# Autodesk Inventor assembly: GPS-Compass_assembly
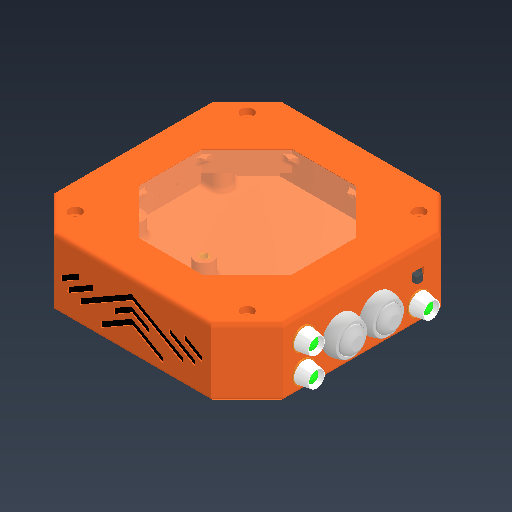
[picture p0: Inventor's stored thumbnail of the model, 512x512]
Saved by Autodesk Inventor 2026.2 (Build 302298000, 298)
## iProperties
Created: 2025-11-19
Part Number: GPS-Compass_assembly
Document SubType Name: Assembly
Designer: MenMe
Author: MenMe
## Documents named in this file (15)
- C:\Users\MenMe\Documents\GitHub\GPS-Compass\_mechanical\GPS-Compass_assembly\GPS-Compass_assembly.iam
- C:\Users\MenMe\Documents\GitHub\GPS-Compass\_mechanical\GPS-Compass_assembly\GPS-Compass_box.ipt
- C:\Users\MenMe\Documents\GitHub\GPS-Compass\_mechanical\GPS-Compass_assembly\GPS-Compass_top.ipt
- C:\Users\MenMe\Documents\GitHub\GPS-Compass\_mechanical\GPS-Compass_assembly\GPS-Compass_plexi.ipt
- C:\Users\MenMe\Documents\GitHub\GPS-Compass\_mechanical\GPS-Compass_assembly\parts\DODGE INSERT M3X4(D5-Dill4.8)\DODGE INSERT M3X4(D5-Dill4.8)\DODGE INSERT M3X4(D5-Dill4.8).ipt
- C:\Users\MenMe\Documents\GitHub\GPS-Compass\_mechanical\GPS-Compass_assembly\parts\ic184-thread\ic184-thread\ic184-thread.ipt
- C:\Users\MenMe\Documents\GitHub\GPS-Compass\_mechanical\GPS-Compass_assembly\parts\Copper Shell LED Indicator Light KL0624\Copper Shell LED Indicator Light KL0624\Copper Shell LED Indicator Light KL0624.ipt
- C:\Users\MenMe\Documents\GitHub\GPS-Compass\_mechanical\GPS-Compass_assembly\parts\EG1201\EG1201\EG1201.ipt
- C:\Users\MenMe\Documents\GitHub\GPS-Compass\_mechanical\GPS-Compass_assembly\parts\antena\antena\antena.ipt
- C:\Users\MenMe\Documents\GitHub\GPS-Compass\_mechanical\PCB_3D_models\GPS-Compass\GPS-Compass\GPS-Compass.ipt
- C:\Users\MenMe\Documents\GitHub\GPS-Compass\_mechanical\PCB_3D_models\GPS-Compass_UI\GPS-Compass_UI\GPS-Compass_UI.ipt
- C:\Users\MenMe\Documents\GitHub\GPS-Compass\_mechanical\PCB_3D_models\GPS-Compass_GNSS\GPS-Compass_GNSS\GPS-Compass_GNSS.ipt
- C:\Users\MenMe\Documents\GitHub\GPS-Compass\_mechanical\PCB_3D_models\GPS-Compass_Arrow\GPS-Compass_Arrow\GPS-Compass_Arrow.ipt
- C:\Users\MenMe\Documents\Inventor\Content Center Files\R2026\en-US\ISO 4762(2)\ISO 4762 - M3 x 12ISO.ipt
- C:\Users\MenMe\Documents\Inventor\Content Center Files\R2026\en-US\ISO 4762(2)\ISO 4762 - M3 x 6ISO.ipt
## Components (36 placed, 14 different names)
1. GPS-Compass_box:1 — Insert:7, Insert:8, Insert:9, Mate:11, Insert:10, Insert:12, Insert:15, Insert:21, Flush:5, Flush:6, Flush:7, Insert:48, Insert:49, Insert:50, Mate:28, Mate:30, Mate:32, Insert:64, Insert:65, Mate:33, Mate:34, Insert:66, Insert:67
2. GPS-Compass_top:1 — Mate:8, Flush:5, Flush:6, Flush:7, Mate:17, Insert:51, Insert:52, Insert:53, Insert:54, Insert:55, Insert:56, Mate:28, Mate:29
3. GPS-Compass_plexi:1 — Mate:8, Mate:17, Mate:29
4. GPS-Compass:1 — Flush:8, Flush:9, Mate:26, Flush:10, Flush:11, Mate:27, Insert:49, Insert:50, Insert:57, Insert:58, Insert:60, Insert:62, Insert:63
5. GPS-Compass_UI:1 — Flush:8, Flush:9, Mate:26
6. GPS-Compass_GNSS:1 — Flush:10, Flush:11, Mate:27, Insert:59, Insert:61
7. GPS-Compass_Arrow:1 — Insert:51, Insert:52
8. Copper Shell LED Indicator Light KL0624:1 — Insert:48
9. EG1201:1 — Mate:30, Mate:32
10. antena:1 — Mate:33, Mate:34
11. ic184-thread:4 — Insert:64
12. ic184-thread:5 — Insert:65
13. Copper Shell LED Indicator Light KL0624:2 — Insert:67
14. Copper Shell LED Indicator Light KL0624:3 — Insert:66
15. ISO 4762 M3 x 12:1 — Insert:53
16. ISO 4762 M3 x 12:2 — Insert:54
17. ISO 4762 M3 x 12:4 — Insert:55
18. ISO 4762 M3 x 12:5 — Insert:56
19. ISO 4762 M3 x 6:1 — Insert:57
20. ISO 4762 M3 x 6:2 — Insert:58
21. ISO 4762 M3 x 6:3 — Insert:59
22. ISO 4762 M3 x 6:4 — Insert:61
23. ISO 4762 M3 x 6:5 — Insert:62
24. ISO 4762 M3 x 6:7 — Insert:63
25. ISO 4762 M3 x 6:8 — Insert:60
26. DODGE INSERT M3X4(D5-Dill4.8):3 — Insert:7
27. DODGE INSERT M3X4(D5-Dill4.8):4 — Insert:8
28. DODGE INSERT M3X4(D5-Dill4.8):5 — Insert:9
29. DODGE INSERT M3X4(D5-Dill4.8):6 — Mate:11
30. DODGE INSERT M3X4(D5-Dill4.8):7 — Insert:10
31. DODGE INSERT M3X4(D5-Dill4.8):9 — Insert:12
32. DODGE INSERT M3X4(D5-Dill4.8):12 — Insert:15
33. DODGE INSERT M3X4(D5-Dill4.8):13
34. DODGE INSERT M3X4(D5-Dill4.8):14
35. DODGE INSERT M3X4(D5-Dill4.8):15
36. DODGE INSERT M3X4(D5-Dill4.8):16 — Insert:21
## Relationships (45: Insert 27, Mate 11, Flush 7)
- Mate:8: GPS-Compass_top:1 ↔ GPS-Compass_plexi:1
- Insert:7: GPS-Compass_box:1 ↔ DODGE INSERT M3X4(D5-Dill4.8):3
- Insert:8: GPS-Compass_box:1 ↔ DODGE INSERT M3X4(D5-Dill4.8):4
- Insert:9: GPS-Compass_box:1 ↔ DODGE INSERT M3X4(D5-Dill4.8):5
- Mate:11: GPS-Compass_box:1 ↔ DODGE INSERT M3X4(D5-Dill4.8):6
- Insert:10: GPS-Compass_box:1 ↔ DODGE INSERT M3X4(D5-Dill4.8):7
- Insert:12: GPS-Compass_box:1 ↔ DODGE INSERT M3X4(D5-Dill4.8):9
- Insert:15: GPS-Compass_box:1 ↔ DODGE INSERT M3X4(D5-Dill4.8):12
- Insert:21: GPS-Compass_box:1 ↔ DODGE INSERT M3X4(D5-Dill4.8):16
- Flush:5: GPS-Compass_box:1 ↔ GPS-Compass_top:1
- Flush:6: GPS-Compass_box:1 ↔ GPS-Compass_top:1
- Flush:7: GPS-Compass_box:1 ↔ GPS-Compass_top:1
- Mate:17: GPS-Compass_top:1 ↔ GPS-Compass_plexi:1
- Insert:48: GPS-Compass_box:1 ↔ Copper Shell LED Indicator Light KL0624:1
- Flush:8: GPS-Compass:1 ↔ GPS-Compass_UI:1
- Flush:9: GPS-Compass:1 ↔ GPS-Compass_UI:1
- Mate:26 (-1 mm): GPS-Compass:1 ↔ GPS-Compass_UI:1
- Flush:10: GPS-Compass:1 ↔ GPS-Compass_GNSS:1
- Flush:11: GPS-Compass:1 ↔ GPS-Compass_GNSS:1
- Mate:27: GPS-Compass:1 ↔ GPS-Compass_GNSS:1
- Insert:49: GPS-Compass_box:1 ↔ GPS-Compass:1
- Insert:50: GPS-Compass_box:1 ↔ GPS-Compass:1
- Insert:51: GPS-Compass_top:1 ↔ GPS-Compass_Arrow:1
- Insert:52: GPS-Compass_top:1 ↔ GPS-Compass_Arrow:1
- Insert:53: GPS-Compass_top:1 ↔ ISO 4762 M3 x 12:1
- Insert:54: GPS-Compass_top:1 ↔ ISO 4762 M3 x 12:2
- Insert:55: GPS-Compass_top:1 ↔ ISO 4762 M3 x 12:4
- Insert:56: GPS-Compass_top:1 ↔ ISO 4762 M3 x 12:5
- Insert:57: GPS-Compass:1 ↔ ISO 4762 M3 x 6:1
- Insert:58: GPS-Compass:1 ↔ ISO 4762 M3 x 6:2
- Insert:59: GPS-Compass_GNSS:1 ↔ ISO 4762 M3 x 6:3
- Insert:60: GPS-Compass:1 ↔ ISO 4762 M3 x 6:8
- Insert:61: GPS-Compass_GNSS:1 ↔ ISO 4762 M3 x 6:4
- Insert:62: GPS-Compass:1 ↔ ISO 4762 M3 x 6:5
- Insert:63: GPS-Compass:1 ↔ ISO 4762 M3 x 6:7
- Mate:28: GPS-Compass_box:1 ↔ GPS-Compass_top:1
- Mate:29: GPS-Compass_top:1 ↔ GPS-Compass_plexi:1
- Mate:30: GPS-Compass_box:1 ↔ EG1201:1
- Mate:32: GPS-Compass_box:1 ↔ EG1201:1
- Insert:64: GPS-Compass_box:1 ↔ ic184-thread:4
- Insert:65: GPS-Compass_box:1 ↔ ic184-thread:5
- Mate:33: GPS-Compass_box:1 ↔ antena:1
- Mate:34: GPS-Compass_box:1 ↔ antena:1
- Insert:66: GPS-Compass_box:1 ↔ Copper Shell LED Indicator Light KL0624:3
- Insert:67: GPS-Compass_box:1 ↔ Copper Shell LED Indicator Light KL0624:2
